# Autodesk Inventor assembly: Pulley
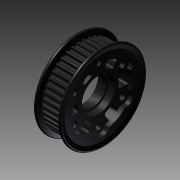
[picture p0: Inventor's stored thumbnail of the model, 180x180]
Saved by Autodesk Inventor 2014 SP1 (Build 180222100, 222)
## iProperties
Created: 2014-01-21
Part Number: Pulley
Document SubType Name: Assembly
Designer: Nick
Author: Nick
## Documents named in this file (2)
- D:\Dropbox\School\PurdueFIRST\PFP Robot\PFP Robot with Cart\Pulley.iam
- D:\Dropbox\School\PurdueFIRST\PFP Robot\PFP Robot with Cart\am-2234_42toothHTDpulleyHalfRev2.ipt
## Components (2 placed, 1 different names)
1. am-2234_42toothHTDpulleyHalfRev2:1 — Insert:1, Insert:2
2. am-2234_42toothHTDpulleyHalfRev2:2 — Insert:1, Insert:2
## Relationships (2: Insert 2)
- Insert:1: am-2234_42toothHTDpulleyHalfRev2:1 ↔ am-2234_42toothHTDpulleyHalfRev2:2
- Insert:2: am-2234_42toothHTDpulleyHalfRev2:1 ↔ am-2234_42toothHTDpulleyHalfRev2:2
